# Autodesk Inventor assembly: cc_unnamed
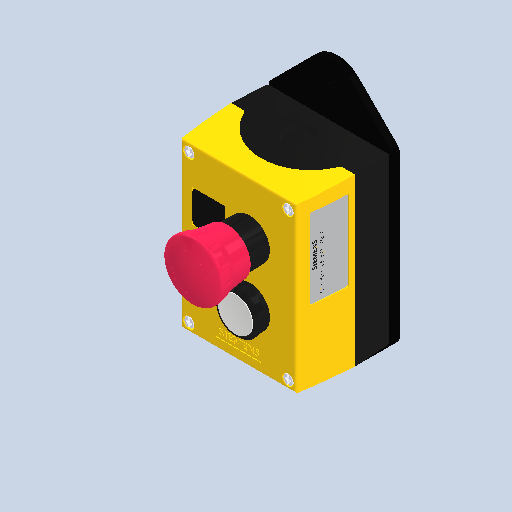
[picture p0: Inventor's stored thumbnail of the model, 512x512]
Saved by Autodesk Inventor 2023 (Build 270158000, 158)
## iProperties
Company: CADClick - www.CADClick.com
Created: 2023-07-21
Part Number: cc_unnamed
Description: STEP AP214
Document SubType Name: Assembly
Designer: chriboehm
Authority: unknown authorization
Mass: 651.868 g
Surface Area: 1101.79 cm^2
Volume: 651.868 cm^3
Density: 1 g/cm^3
Preprocessor: Spatial InterOp 3D postprocessed
Title: cctmp_F6C4ABE3-F9DC-40F7-ADFA-5E338C1169B7_2023_07_21_14_44_37_0671..stp
Author: SIEMENS A&D
Revision Number: NONE
## Documents named in this file (5)
- C:\work\robots\butler_2.0\body_model\parts\emergancy_stop\G_IC03_XX_12648V.iam
- C:\work\robots\butler_2.0\body_model\parts\emergancy_stop\2023_07_21_14_44_37_0611.ipt
- C:\work\robots\butler_2.0\body_model\parts\emergancy_stop\2023_07_21_14_44_37_0603.ipt
- C:\work\robots\butler_2.0\body_model\parts\emergancy_stop\G_IC03_XX_13055V.iam
- C:\work\robots\butler_2.0\body_model\parts\emergancy_stop\mount.ipt
## Components (4 placed, 4 different names)
1. 2023_07_21_14_44_37_0611 — Mate:3, Mate:4
2. 2023_07_21_14_44_37_0603 — Mate:1, Mate:2, Mate:3, Mate:4, Flush:1, Flush:2
3. G_IC03_XX_13055V:1 [sub-assembly] — Mate:1, Mate:2
4. mount:1 — Flush:1, Flush:2
## Relationships (6: Mate 4, Flush 2)
- Mate:1: 2023_07_21_14_44_37_0603 ↔ G_IC03_XX_13055V:1
- Mate:2: 2023_07_21_14_44_37_0603 ↔ G_IC03_XX_13055V:1
- Mate:3: 2023_07_21_14_44_37_0611 ↔ 2023_07_21_14_44_37_0603
- Mate:4: 2023_07_21_14_44_37_0611 ↔ 2023_07_21_14_44_37_0603
- Flush:1: 2023_07_21_14_44_37_0603 ↔ mount:1
- Flush:2: 2023_07_21_14_44_37_0603 ↔ mount:1
